# Autodesk Inventor assembly: YAxis_Carriage
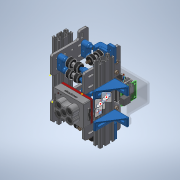
[picture p0: Inventor's stored thumbnail of the model, 180x180]
Saved by Autodesk Inventor 2021 (Build 250183000, 183)
## iProperties
Created: 2021-02-02
Part Number: YAxis_Carriage
Document SubType Name: Assembly
Designer: Jorian Brusind
Author: Jorian Brusind
## Documents named in this file (22)
- C:\Users\Jorian Brusind\Documents\GitHub\PersonalProjects\HyperRail\Inventor Files\YAxis_Carriage.iam
- C:\Users\Jorian Brusind\Documents\GitHub\PersonalProjects\HyperRail\Inventor Files\SmallBelt_Pulley.ipt
- C:\Users\Jorian Brusind\Documents\GitHub\PersonalProjects\Inventor Projects\Useful models\Metric bolt\Bolt M3 30mm.ipt
- C:\Users\Jorian Brusind\Documents\GitHub\PersonalProjects\HyperRail\Inventor Files\small_belt_loop.ipt
- C:\Users\Jorian Brusind\Documents\GitHub\PersonalProjects\HyperRail\PCB Files\Integrated Stepper Motor Driver\ExportSTEP\Main.iam
- C:\Users\Jorian Brusind\Documents\GitHub\PersonalProjects\HyperRail\Inventor Files\rededge-micasense-1.snapshot.3\PND_CAM_MSRE.ipt
- C:\Users\Jorian Brusind\Documents\GitHub\PersonalProjects\HyperRail\Inventor Files\NEMA17_Shroud.ipt
- C:\Users\Jorian Brusind\Documents\GitHub\PersonalProjects\HyperRail\Inventor Files\Buffer.iam
- C:\Users\Jorian Brusind\Documents\GitHub\PersonalProjects\HyperRail\Inventor Files\X_CarriageR_V2_1.iam
- C:\Users\Jorian Brusind\Documents\GitHub\PersonalProjects\HyperRail\Inventor Files\X_Carriage_V2_1.iam
- C:\Users\Jorian Brusind\Documents\GitHub\PersonalProjects\Inventor Projects\Useful models\8020_Sets\IPT_20_Series\IPT_20_Series\20-2040_200mm.ipt
- C:\Users\Jorian Brusind\Documents\GitHub\PersonalProjects\HyperRail\Inventor Files\10mm_Idle_Pulley_3M.ipt
- C:\Users\Jorian Brusind\Documents\GitHub\PersonalProjects\HyperRail\Inventor Files\McMaster Files\Hex Standoffs\95947A725_Aluminum Female Threaded Hex Standoff.ipt
- C:\Users\Jorian Brusind\Documents\GitHub\PersonalProjects\Inventor Projects\Useful models\Metric bolt\Bolt M5 45mm.ipt
- C:\Users\Jorian Brusind\Documents\GitHub\PersonalProjects\HyperRail\Inventor Files\nema17-x-40-1.snapshot.7\NEMA17 x 40.ipt
- C:\Users\Jorian Brusind\Documents\GitHub\PersonalProjects\HyperRail\Inventor Files\RightAngle_Bracket.ipt
- C:\Users\Jorian Brusind\Documents\GitHub\PersonalProjects\HyperRail\Inventor Files\X_Carriage_Plate.ipt
- C:\Users\Jorian Brusind\Documents\GitHub\PersonalProjects\HyperRail\Inventor Files\11mm_BearingWheel.ipt
- C:\Users\Jorian Brusind\Documents\GitHub\PersonalProjects\HyperRail\Inventor Files\30mm_HeatInsertSpacer.ipt
- C:\Users\Jorian Brusind\Documents\GitHub\PersonalProjects\Inventor Projects\Useful models\Metric bolt\Bolt M5 25mm.ipt
- C:\Users\Jorian Brusind\Documents\GitHub\PersonalProjects\HyperRail\Inventor Files\Belt_Clamp.ipt
- C:\Users\Jorian Brusind\Documents\GitHub\PersonalProjects\HyperRail\Inventor Files\4mm_Roller_Spacer_extended.ipt
## Components (53 placed, 21 different names)
1. SmallBelt_Pulley:1 — Mate:37, Flush:94, Mate:208, Flush:102, Flush:103
2. small_belt_loop:1 — Mate:37, Mate:213, Angle:1
3. Main:1 [sub-assembly] — Mate:209, Mate:210, Mate:211
4. PND_CAM_MSRE:1 — Mate:188, Flush:95, Mate:189
5. 20-2040_200mm:1 — Flush:74, Flush:75, Mate:151, Mate:188, Mate:228, Mate:229, Flush:114
6. 20-2040_200mm:2 — Flush:74, Flush:75, Mate:155, Mate:156, Mate:160, Mate:174, Flush:95, Mate:223, Mate:224, Mate:227, Mate:296, Flush:126, Flush:127, Flush:128, Mate:297, Flush:129, Flush:130
7. X_Carriage_V2_1:3 [sub-assembly] — Mate:160, Mate:190, Mate:193, Mate:198, Mate:199, Mate:205, Flush:103, Flush:106, Flush:107, Flush:112, Mate:240, Mate:241, Mate:246, Mate:260, Mate:261, Mate:281, Mate:286, Mate:290, Mate:293, Mate:302, Mate:303, Mate:304, Flush:130, Mate:313, Mate:315
8. Bolt M3 30mm:2 — Mate:183, Mate:184, Mate:219
9. X_CarriageR_V2_1:1 [sub-assembly] — Mate:174, Mate:189, Mate:195, Mate:197, Mate:203, Mate:204, Mate:217, Flush:109, Mate:237, Mate:238, Flush:112, Mate:256, Mate:258, Mate:259, Mate:277, Mate:280, Mate:282, Mate:283, Mate:288, Mate:295, Mate:298, Mate:301, Mate:316
10. 10mm_Idle_Pulley_3M:1 — Flush:93, Mate:222
11. 10mm_Idle_Pulley_3M:2 — Flush:91, Mate:220
12. 10mm_Idle_Pulley_3M:3 — Flush:92, Mate:221
13. 10mm_Idle_Pulley_3M:4 — Flush:91, Flush:92, Flush:93, Flush:94, Mate:183, Mate:184
14. 95947A725_Aluminum Female Threaded Hex Standoff:1 — Mate:190, Mate:245
15. 95947A725_Aluminum Female Threaded Hex Standoff:2 — Mate:193, Mate:242
16. 95947A725_Aluminum Female Threaded Hex Standoff:3 — Mate:195, Mate:254, Mate:256
17. 95947A725_Aluminum Female Threaded Hex Standoff:4 — Mate:197, Mate:253, Mate:255
18. Bolt M5 45mm:1 — Flush:96, Flush:101, Mate:242, Mate:243, Mate:246
19. Bolt M5 45mm:2 — Mate:198, Flush:97
20. Bolt M5 45mm:3 — Flush:100, Flush:101, Mate:254, Mate:299, Mate:308
21. Bolt M5 45mm:4 — Flush:100, Mate:253, Mate:300
22. Bolt M5 45mm:5 — Flush:96, Mate:245, Mate:305
23. Bolt M5 45mm:6 — Mate:203, Flush:98, Flush:99
24. Bolt M5 45mm:7 — Mate:204, Flush:98, Mate:255
25. Bolt M5 45mm:8 — Mate:199, Flush:97, Flush:99, Mate:205
26. NEMA17 x 40:1 — Mate:208, Mate:209, Mate:210, Mate:211, Mate:213, Flush:102, Mate:214, Mate:215, Mate:216
27. NEMA17_Shroud:1 — Mate:214, Mate:215, Mate:216, Mate:217, Mate:219, Mate:220, Mate:221, Mate:222, Angle:1, Mate:225, Mate:226, Flush:104, Flush:105, Mate:227
28. RightAngle_Bracket:1 — Mate:224, Mate:226, Flush:104
29. RightAngle_Bracket:2 — Mate:223, Mate:225, Flush:105
30. X_Carriage_Plate:1 — Mate:228, Flush:106, Flush:107, Flush:108, Mate:243, Mate:309, Mate:311
31. X_Carriage_Plate:2 — Mate:229, Flush:108, Flush:109, Flush:114, Mate:310, Mate:312
32. 11mm_BearingWheel:1 — Mate:241, Mate:306
33. 11mm_BearingWheel:2 — Mate:240, Mate:317
34. 11mm_BearingWheel:3 — Mate:237, Mate:262, Mate:314
35. 11mm_BearingWheel:4 — Mate:238, Mate:307, Mate:318
36. 95947A725_Aluminum Female Threaded Hex Standoff:5 — Flush:117, Mate:261
37. 95947A725_Aluminum Female Threaded Hex Standoff:6 — Mate:259, Flush:115, Mate:262
38. 95947A725_Aluminum Female Threaded Hex Standoff:7 — Flush:116, Flush:117, Mate:260
39. 95947A725_Aluminum Female Threaded Hex Standoff:8 — Mate:258, Flush:115, Flush:116, Mate:277
40. 30mm_HeatInsertSpacer:2 — Mate:281, Flush:118, Mate:282
41. 30mm_HeatInsertSpacer:3 — Mate:280, Flush:118
42. Bolt M5 25mm:2 — Mate:283, Mate:295
43. Bolt M5 25mm:4 — Mate:290
44. Bolt M5 25mm:5 — Mate:288
45. Bolt M5 25mm:6 — Mate:286, Mate:293
46. Buffer:1 [sub-assembly] — Mate:296, Flush:126, Flush:127
47. Buffer:2 [sub-assembly] — Flush:128, Mate:297, Flush:129, Mate:298
48. Belt_Clamp:1 — Mate:299, Mate:300, Mate:301
49. Belt_Clamp:2 — Mate:302, Mate:303, Mate:304
50. 4mm_Roller_Spacer_extended:1 — Mate:307, Mate:312, Mate:314, Mate:318
51. 4mm_Roller_Spacer_extended:2 — Mate:308, Mate:310, Mate:316, Flush:131
52. 4mm_Roller_Spacer_extended:3 — Mate:306, Mate:311, Mate:313, Mate:317
53. 4mm_Roller_Spacer_extended:4 — Mate:305, Mate:309, Mate:315, Flush:131
## Relationships (125: Mate 89, Flush 35, Angle 1)
- Mate:37 (2 mm): SmallBelt_Pulley:1 ↔ small_belt_loop:1
- Flush:74: 20-2040_200mm:1 ↔ 20-2040_200mm:2
- Flush:75: 20-2040_200mm:1 ↔ 20-2040_200mm:2
- Mate:151: 20-2040_200mm:1
- Mate:155: 20-2040_200mm:2
- Mate:156: 20-2040_200mm:2
- Mate:160: 20-2040_200mm:2 ↔ X_Carriage_V2_1:3
- Mate:174: 20-2040_200mm:2 ↔ X_CarriageR_V2_1:1
- Flush:91: 10mm_Idle_Pulley_3M:2 ↔ 10mm_Idle_Pulley_3M:4
- Flush:92: 10mm_Idle_Pulley_3M:3 ↔ 10mm_Idle_Pulley_3M:4
- Flush:93: 10mm_Idle_Pulley_3M:1 ↔ 10mm_Idle_Pulley_3M:4
- Flush:94: SmallBelt_Pulley:1 ↔ 10mm_Idle_Pulley_3M:4
- Mate:183: Bolt M3 30mm:2 ↔ 10mm_Idle_Pulley_3M:4
- Mate:184: Bolt M3 30mm:2 ↔ 10mm_Idle_Pulley_3M:4
- Mate:188 (20 mm): PND_CAM_MSRE:1 ↔ 20-2040_200mm:1
- Flush:95: PND_CAM_MSRE:1 ↔ 20-2040_200mm:2
- Mate:189 (0.5 mm): PND_CAM_MSRE:1 ↔ X_CarriageR_V2_1:1
- Mate:190: X_Carriage_V2_1:3 ↔ 95947A725_Aluminum Female Threaded Hex Standoff:1
- Mate:193: X_Carriage_V2_1:3 ↔ 95947A725_Aluminum Female Threaded Hex Standoff:2
- Mate:195: X_CarriageR_V2_1:1 ↔ 95947A725_Aluminum Female Threaded Hex Standoff:3
- Mate:197: X_CarriageR_V2_1:1 ↔ 95947A725_Aluminum Female Threaded Hex Standoff:4
- Mate:198: X_Carriage_V2_1:3 ↔ Bolt M5 45mm:2
- Mate:199: X_Carriage_V2_1:3 ↔ Bolt M5 45mm:8
- Flush:96: Bolt M5 45mm:1 ↔ Bolt M5 45mm:5
- Flush:97: Bolt M5 45mm:2 ↔ Bolt M5 45mm:8
- Mate:203: X_CarriageR_V2_1:1 ↔ Bolt M5 45mm:6
- Mate:204: X_CarriageR_V2_1:1 ↔ Bolt M5 45mm:7
- Flush:98: Bolt M5 45mm:6 ↔ Bolt M5 45mm:7
- Flush:99: Bolt M5 45mm:6 ↔ Bolt M5 45mm:8
- Mate:205: X_Carriage_V2_1:3 ↔ Bolt M5 45mm:8
- Flush:100: Bolt M5 45mm:3 ↔ Bolt M5 45mm:4
- Flush:101: Bolt M5 45mm:1 ↔ Bolt M5 45mm:3
- Mate:208: SmallBelt_Pulley:1 ↔ NEMA17 x 40:1
- Mate:209: Main:1 ↔ NEMA17 x 40:1
- Mate:210: Main:1 ↔ NEMA17 x 40:1
- Mate:211 (8 mm): Main:1 ↔ NEMA17 x 40:1
- Mate:213: small_belt_loop:1 ↔ NEMA17 x 40:1
- Flush:102: SmallBelt_Pulley:1 ↔ NEMA17 x 40:1
- Flush:103: SmallBelt_Pulley:1 ↔ X_Carriage_V2_1:3
- Mate:214: NEMA17 x 40:1 ↔ NEMA17_Shroud:1
- Mate:215: NEMA17 x 40:1 ↔ NEMA17_Shroud:1
- Mate:216: NEMA17 x 40:1 ↔ NEMA17_Shroud:1
- Mate:217 (3 mm): X_CarriageR_V2_1:1 ↔ NEMA17_Shroud:1
- Mate:219: Bolt M3 30mm:2 ↔ NEMA17_Shroud:1
- Mate:220: 10mm_Idle_Pulley_3M:2 ↔ NEMA17_Shroud:1
- Mate:221: 10mm_Idle_Pulley_3M:3 ↔ NEMA17_Shroud:1
- Mate:222: 10mm_Idle_Pulley_3M:1 ↔ NEMA17_Shroud:1
- Angle:1 (0 deg): small_belt_loop:1 ↔ NEMA17_Shroud:1
- Mate:223: 20-2040_200mm:2 ↔ RightAngle_Bracket:2
- Mate:224: 20-2040_200mm:2 ↔ RightAngle_Bracket:1
- Mate:225: NEMA17_Shroud:1 ↔ RightAngle_Bracket:2
- Mate:226: NEMA17_Shroud:1 ↔ RightAngle_Bracket:1
- Flush:104: NEMA17_Shroud:1 ↔ RightAngle_Bracket:1
- Flush:105: NEMA17_Shroud:1 ↔ RightAngle_Bracket:2
- Mate:227: 20-2040_200mm:2 ↔ NEMA17_Shroud:1
- Mate:228: 20-2040_200mm:1 ↔ X_Carriage_Plate:1
- Flush:106: X_Carriage_V2_1:3 ↔ X_Carriage_Plate:1
- Flush:107: X_Carriage_V2_1:3 ↔ X_Carriage_Plate:1
- Mate:229: 20-2040_200mm:1 ↔ X_Carriage_Plate:2
- Flush:108: X_Carriage_Plate:1 ↔ X_Carriage_Plate:2
- Flush:109: X_CarriageR_V2_1:1 ↔ X_Carriage_Plate:2
- [Flush]: 11mm_BearingWheel:1 ↔ 11mm_BearingWheel:2
- [Flush]: 11mm_BearingWheel:3 ↔ 11mm_BearingWheel:4
- Mate:237: X_CarriageR_V2_1:1 ↔ 11mm_BearingWheel:3
- Mate:238: X_CarriageR_V2_1:1 ↔ 11mm_BearingWheel:4
- Flush:112: X_Carriage_V2_1:3 ↔ X_CarriageR_V2_1:1
- Mate:240: X_Carriage_V2_1:3 ↔ 11mm_BearingWheel:2
- Mate:241: X_Carriage_V2_1:3 ↔ 11mm_BearingWheel:1
- Mate:242: 95947A725_Aluminum Female Threaded Hex Standoff:2 ↔ Bolt M5 45mm:1
- Mate:243: Bolt M5 45mm:1 ↔ X_Carriage_Plate:1
- Flush:114: 20-2040_200mm:1 ↔ X_Carriage_Plate:2
- Mate:245: 95947A725_Aluminum Female Threaded Hex Standoff:1 ↔ Bolt M5 45mm:5
- Mate:246: X_Carriage_V2_1:3 ↔ Bolt M5 45mm:1
- Mate:253: 95947A725_Aluminum Female Threaded Hex Standoff:4 ↔ Bolt M5 45mm:4
- Mate:254: 95947A725_Aluminum Female Threaded Hex Standoff:3 ↔ Bolt M5 45mm:3
- Mate:255: 95947A725_Aluminum Female Threaded Hex Standoff:4 ↔ Bolt M5 45mm:7
- Mate:256: X_CarriageR_V2_1:1 ↔ 95947A725_Aluminum Female Threaded Hex Standoff:3
- Mate:258: X_CarriageR_V2_1:1 ↔ 95947A725_Aluminum Female Threaded Hex Standoff:8
- Mate:259: X_CarriageR_V2_1:1 ↔ 95947A725_Aluminum Female Threaded Hex Standoff:6
- Flush:115: 95947A725_Aluminum Female Threaded Hex Standoff:6 ↔ 95947A725_Aluminum Female Threaded Hex Standoff:8
- Flush:116: 95947A725_Aluminum Female Threaded Hex Standoff:7 ↔ 95947A725_Aluminum Female Threaded Hex Standoff:8
- Flush:117: 95947A725_Aluminum Female Threaded Hex Standoff:5 ↔ 95947A725_Aluminum Female Threaded Hex Standoff:7
- Mate:260: X_Carriage_V2_1:3 ↔ 95947A725_Aluminum Female Threaded Hex Standoff:7
- Mate:261: X_Carriage_V2_1:3 ↔ 95947A725_Aluminum Female Threaded Hex Standoff:5
- Mate:262: 11mm_BearingWheel:3 ↔ 95947A725_Aluminum Female Threaded Hex Standoff:6
- Mate:277: X_CarriageR_V2_1:1 ↔ 95947A725_Aluminum Female Threaded Hex Standoff:8
- Mate:280: X_CarriageR_V2_1:1 ↔ 30mm_HeatInsertSpacer:3
- Mate:281: X_Carriage_V2_1:3 ↔ 30mm_HeatInsertSpacer:2
- Flush:118: 30mm_HeatInsertSpacer:2 ↔ 30mm_HeatInsertSpacer:3
- Mate:282 (2.5 mm): X_CarriageR_V2_1:1 ↔ 30mm_HeatInsertSpacer:2
- Mate:283: X_CarriageR_V2_1:1 ↔ Bolt M5 25mm:2
- Mate:286: X_Carriage_V2_1:3 ↔ Bolt M5 25mm:6
- Mate:288: X_CarriageR_V2_1:1 ↔ Bolt M5 25mm:5
- Mate:290: X_Carriage_V2_1:3 ↔ Bolt M5 25mm:4
- Mate:293: X_Carriage_V2_1:3 ↔ Bolt M5 25mm:6
- Mate:295: X_CarriageR_V2_1:1 ↔ Bolt M5 25mm:2
- Mate:296: 20-2040_200mm:2 ↔ Buffer:1
- Flush:126: 20-2040_200mm:2 ↔ Buffer:1
- Flush:127: 20-2040_200mm:2 ↔ Buffer:1
- Flush:128: 20-2040_200mm:2 ↔ Buffer:2
- Mate:297: 20-2040_200mm:2 ↔ Buffer:2
- Flush:129: 20-2040_200mm:2 ↔ Buffer:2
- Mate:298 (5 mm): X_CarriageR_V2_1:1 ↔ Buffer:2
- Mate:299: Bolt M5 45mm:3 ↔ Belt_Clamp:1
- Mate:300: Bolt M5 45mm:4 ↔ Belt_Clamp:1
- Mate:301 (1 mm): X_CarriageR_V2_1:1 ↔ Belt_Clamp:1
- Mate:302: X_Carriage_V2_1:3 ↔ Belt_Clamp:2
- Mate:303: X_Carriage_V2_1:3 ↔ Belt_Clamp:2
- Mate:304 (1 mm): X_Carriage_V2_1:3 ↔ Belt_Clamp:2
- Flush:130: 20-2040_200mm:2 ↔ X_Carriage_V2_1:3
- Mate:305: Bolt M5 45mm:5 ↔ 4mm_Roller_Spacer_extended:4
- Mate:306: 11mm_BearingWheel:1 ↔ 4mm_Roller_Spacer_extended:3
- Mate:307: 11mm_BearingWheel:4 ↔ 4mm_Roller_Spacer_extended:1
- Mate:308: Bolt M5 45mm:3 ↔ 4mm_Roller_Spacer_extended:2
- Mate:309: X_Carriage_Plate:1 ↔ 4mm_Roller_Spacer_extended:4
- Mate:310: X_Carriage_Plate:2 ↔ 4mm_Roller_Spacer_extended:2
- Mate:311: X_Carriage_Plate:1 ↔ 4mm_Roller_Spacer_extended:3
- Mate:312: X_Carriage_Plate:2 ↔ 4mm_Roller_Spacer_extended:1
- Mate:313: X_Carriage_V2_1:3 ↔ 4mm_Roller_Spacer_extended:3
- Mate:314: 11mm_BearingWheel:3 ↔ 4mm_Roller_Spacer_extended:1
- Mate:315: X_Carriage_V2_1:3 ↔ 4mm_Roller_Spacer_extended:4
- Mate:316: X_CarriageR_V2_1:1 ↔ 4mm_Roller_Spacer_extended:2
- Flush:131: 4mm_Roller_Spacer_extended:2 ↔ 4mm_Roller_Spacer_extended:4
- Mate:317: 11mm_BearingWheel:2 ↔ 4mm_Roller_Spacer_extended:3
- Mate:318: 11mm_BearingWheel:4 ↔ 4mm_Roller_Spacer_extended:1
## Named parameters: d422_d7 = 0 mm
